# Autodesk Inventor assembly: GPS.ipt
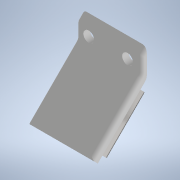
[picture p0: Inventor's stored thumbnail of the model, 180x180]
Saved by Autodesk Inventor 2022 (Build 260153000, 153)
## iProperties
Created: 2022-05-03
Part Number: GPS.ipt
Document SubType Name: Assembly
Designer: Кочетов.А.И.
Author: Кочетов.А.И.
## Documents named in this file (3)
- C:\Users\BornO\Documents\Inventor\БАСУ\GPS.ipt.iam
- C:\Users\BornO\Documents\Inventor\БАСУ\Держатель GPS.ipt
- C:\Users\BornO\Documents\Inventor\БАСУ\Антена GPS.ipt
## Components (2 placed, 2 different names)
1. Держатель GPS:1 — Совмещение:1, Совмещение:2, Заподлицо:1, Совмещение:3, Совмещение:4, Совмещение:5
2. Антена GPS:1 — Совмещение:3, Совмещение:4, Совмещение:5
## Relationships (6: Mate 5, Flush 1)
- Совмещение:1 [Mate]: Держатель GPS:1
- Совмещение:2 [Mate]: Держатель GPS:1
- Заподлицо:1 [Flush]: Держатель GPS:1
- Совмещение:3 [Mate]: Держатель GPS:1 ↔ Антена GPS:1
- Совмещение:4 [Mate]: Держатель GPS:1 ↔ Антена GPS:1
- Совмещение:5 [Mate]: Держатель GPS:1 ↔ Антена GPS:1
